# Autodesk Inventor assembly: gears
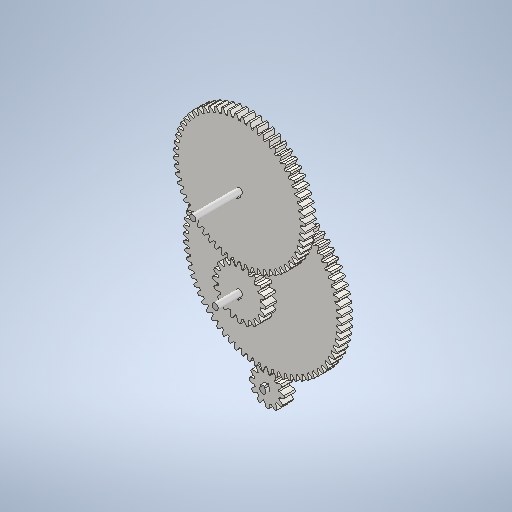
[picture p0: Inventor's stored thumbnail of the model, 512x512]
Saved by Autodesk Inventor 2025 (Build 290162010, 162A)
## iProperties
Created: 2024-07-26
Part Number: gears
Document SubType Name: Assembly
Designer: saees
Author: saees
## Documents named in this file (5)
- C:\Users\saees\OneDrive\Documents\Inventor\gears.iam
- C:\Users\saees\OneDrive\Documents\Inventor\gears\Design Accelerator\Spur Gears3.iam
- C:\Users\saees\OneDrive\Documents\Inventor\gears\Design Accelerator\Spur Gears4.iam
- C:\Users\saees\OneDrive\Documents\Inventor\shaft1.ipt
- C:\Users\saees\OneDrive\Documents\Inventor\shaft2.ipt
## Components (5 placed, 3 different names)
1. Spur Gears:3 [sub-assembly] — Mate:3, Mate:4, Mate:6, Mate:8
2. Spur Gears:4 [sub-assembly] — Mate:1, Mate:2, Mate:5, Mate:7
3. shaft1:1 — Mate:1, Mate:2
4. shaft1:2 — Mate:3, Mate:4
5. shaft2:1 — Mate:5, Mate:6, Mate:7, Mate:8
## Relationships (8: Mate 8)
- Mate:1: Spur Gears:4 ↔ shaft1:1
- Mate:2: Spur Gears:4 ↔ shaft1:1
- Mate:3: Spur Gears:3 ↔ shaft1:2
- Mate:4: Spur Gears:3 ↔ shaft1:2
- Mate:5: Spur Gears:4 ↔ shaft2:1
- Mate:6: Spur Gears:3 ↔ shaft2:1
- Mate:7: Spur Gears:4 ↔ shaft2:1
- Mate:8: Spur Gears:3 ↔ shaft2:1
